# Autodesk Inventor assembly: ASSEMBLY_Main
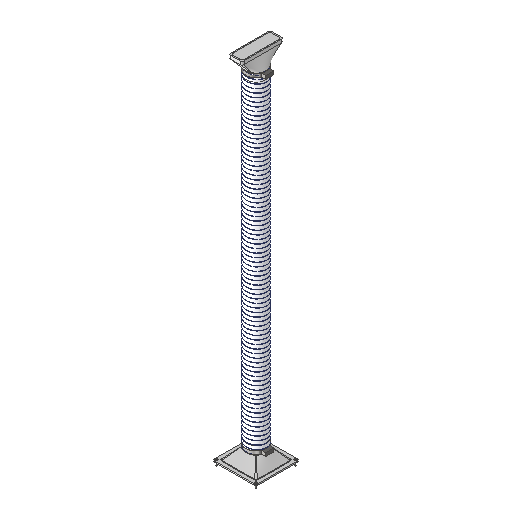
[picture p0: Inventor's stored thumbnail of the model, 512x512]
Saved by Autodesk Inventor 2025 (Build 290162010, 162A)
## iProperties
Created: 2024-10-12
Part Number: ASSEMBLY_Main
Document SubType Name: Assembly
Designer: User
Author: User
## Documents named in this file (9)
- D:\_ANDRZEJ_LACZEWSKI\_OTHER\MECH - Air Purifier Based Soldering Fume Extractor\MCAD\1_REV1\ASSEMBLY_MAIN_REVA\ASSEMBLY_Main.iam
- D:\_ANDRZEJ_LACZEWSKI\_OTHER\MECH - Air Purifier Based Soldering Fume Extractor\MCAD\1_REV1\ASSEMBLY_MAIN_REVA\3DP_PLA_Air_Purifier_60mm_Pipe_Mount.ipt
- D:\_ANDRZEJ_LACZEWSKI\_OTHER\MECH - Air Purifier Based Soldering Fume Extractor\MCAD\1_REV1\__COTS_PARTS\COTS_GENERIC_60mm_PUR_Suction_Hose.ipt
- D:\_ANDRZEJ_LACZEWSKI\_OTHER\MECH - Air Purifier Based Soldering Fume Extractor\MCAD\1_REV1\__COTS_PARTS\COTS_GENERIC_60mm_Hose_Clamp.ipt
- D:\_ANDRZEJ_LACZEWSKI\_OTHER\MECH - Air Purifier Based Soldering Fume Extractor\MCAD\1_REV1\ASSEMBLY_MAIN_REVA\3DP_PLA_Air_Funnel.ipt
- D:\_ANDRZEJ_LACZEWSKI\_OTHER\MECH - Air Purifier Based Soldering Fume Extractor\MCAD\1_REV1\ASSEMBLY_MAIN_REVA\3DP_PLA_Air_Funnel_Grid.ipt
- D:\_ANDRZEJ_LACZEWSKI\_OTHER\MECH - Air Purifier Based Soldering Fume Extractor\MCAD\1_REV1\__CONTENT_CENTER_PARTS\en-US\DIN 125-2  A\DIN 125-2 - A 3,2A.ipt
- D:\_ANDRZEJ_LACZEWSKI\_OTHER\MECH - Air Purifier Based Soldering Fume Extractor\MCAD\1_REV1\__CONTENT_CENTER_PARTS\en-US\ISO 7380-1\ISO 7380-1 - M3 x 16.ipt
- D:\_ANDRZEJ_LACZEWSKI\_OTHER\MECH - Air Purifier Based Soldering Fume Extractor\MCAD\1_REV1\__CONTENT_CENTER_PARTS\en-US\DIN 934\DIN 934 - M3 x 0,5.ipt
## Components (22 placed, 8 different names)
1. 3DP_PLA_Air_Purifier_60mm_Pipe_Mount:1 — Mate:1, Mate:4, Flush:3, Angle:1, Mate:41, Mate:42, Mate:43, Mate:44, Mate:45, Mate:46, Mate:47, Mate:48, Mate:49, Mate:50, Mate:51, Mate:52, Mate:53, Mate:54, Mate:55, Mate:56, Mate:57
2. COTS_GENERIC_60mm_PUR_Suction_Hose:1 — Mate:1, Mate:4, Mate:37, Mate:38, Flush:1, Flush:2, Mate:39, Mate:40
3. COTS_GENERIC_60mm_Hose_Clamp:1 — Mate:37, Flush:2
4. COTS_GENERIC_60mm_Hose_Clamp:2 — Mate:38, Flush:1
5. 3DP_PLA_Air_Funnel:1 — Mate:39, Mate:40, Angle:1, Flush:4
6. 3DP_PLA_Air_Funnel_Grid:1 — Flush:4
7. DIN 934 - replaced by DIN EN 24032/28673/28674 M3:4 — Insert:8
8. DIN 934 - replaced by DIN EN 24032/28673/28674 M3:3 — Insert:7
9. DIN 934 - replaced by DIN EN 24032/28673/28674 M3:2 — Insert:6
10. DIN 125-2 A A 3,2:8 — Mate:56, Mate:57, Insert:8
11. DIN 125-2 A A 3,2:7 — Mate:54, Mate:55, Insert:7
12. DIN 125-2 A A 3,2:6 — Mate:52, Mate:53, Insert:6
13. ISO 7380-1 M3 x 16:4 — Insert:4
14. ISO 7380-1 M3 x 16:3 — Insert:3
15. ISO 7380-1 M3 x 16:2 — Insert:2
16. DIN 125-2 A A 3,2:5 — Mate:48, Mate:49, Insert:4
17. DIN 125-2 A A 3,2:4 — Mate:46, Mate:47, Insert:3
18. DIN 125-2 A A 3,2:3 — Mate:44, Mate:45, Insert:2
19. DIN 934 - replaced by DIN EN 24032/28673/28674 M3:1 — Insert:5
20. DIN 125-2 A A 3,2:2 — Mate:50, Mate:51, Insert:5
21. ISO 7380-1 M3 x 16:1 — Insert:1
22. DIN 125-2 A A 3,2:1 — Mate:42, Mate:43, Insert:1
## Relationships (36: Mate 23, Insert 8, Flush 4, Angle 1)
- Mate:1: 3DP_PLA_Air_Purifier_60mm_Pipe_Mount:1 ↔ COTS_GENERIC_60mm_PUR_Suction_Hose:1
- Mate:4 (-25 mm): 3DP_PLA_Air_Purifier_60mm_Pipe_Mount:1 ↔ COTS_GENERIC_60mm_PUR_Suction_Hose:1
- Mate:37: COTS_GENERIC_60mm_PUR_Suction_Hose:1 ↔ COTS_GENERIC_60mm_Hose_Clamp:1
- Mate:38: COTS_GENERIC_60mm_PUR_Suction_Hose:1 ↔ COTS_GENERIC_60mm_Hose_Clamp:2
- Flush:1: COTS_GENERIC_60mm_PUR_Suction_Hose:1 ↔ COTS_GENERIC_60mm_Hose_Clamp:2
- Flush:2: COTS_GENERIC_60mm_PUR_Suction_Hose:1 ↔ COTS_GENERIC_60mm_Hose_Clamp:1
- Flush:3: 3DP_PLA_Air_Purifier_60mm_Pipe_Mount:1
- Mate:39: COTS_GENERIC_60mm_PUR_Suction_Hose:1 ↔ 3DP_PLA_Air_Funnel:1
- Mate:40 (-25 mm): COTS_GENERIC_60mm_PUR_Suction_Hose:1 ↔ 3DP_PLA_Air_Funnel:1
- Angle:1 (0 deg): 3DP_PLA_Air_Purifier_60mm_Pipe_Mount:1 ↔ 3DP_PLA_Air_Funnel:1
- Flush:4: 3DP_PLA_Air_Funnel:1 ↔ 3DP_PLA_Air_Funnel_Grid:1
- Mate:41 (-500 mm): 3DP_PLA_Air_Purifier_60mm_Pipe_Mount:1
- Mate:42: 3DP_PLA_Air_Purifier_60mm_Pipe_Mount:1 ↔ DIN 125-2 A A 3,2:1
- Mate:43: 3DP_PLA_Air_Purifier_60mm_Pipe_Mount:1 ↔ DIN 125-2 A A 3,2:1
- Mate:44: 3DP_PLA_Air_Purifier_60mm_Pipe_Mount:1 ↔ DIN 125-2 A A 3,2:3
- Mate:45: 3DP_PLA_Air_Purifier_60mm_Pipe_Mount:1 ↔ DIN 125-2 A A 3,2:3
- Mate:46: 3DP_PLA_Air_Purifier_60mm_Pipe_Mount:1 ↔ DIN 125-2 A A 3,2:4
- Mate:47: 3DP_PLA_Air_Purifier_60mm_Pipe_Mount:1 ↔ DIN 125-2 A A 3,2:4
- Mate:48: 3DP_PLA_Air_Purifier_60mm_Pipe_Mount:1 ↔ DIN 125-2 A A 3,2:5
- Mate:49: 3DP_PLA_Air_Purifier_60mm_Pipe_Mount:1 ↔ DIN 125-2 A A 3,2:5
- Insert:1: ISO 7380-1 M3 x 16:1 ↔ DIN 125-2 A A 3,2:1
- Insert:2: ISO 7380-1 M3 x 16:2 ↔ DIN 125-2 A A 3,2:3
- Insert:3: ISO 7380-1 M3 x 16:3 ↔ DIN 125-2 A A 3,2:4
- Insert:4: ISO 7380-1 M3 x 16:4 ↔ DIN 125-2 A A 3,2:5
- Mate:50: 3DP_PLA_Air_Purifier_60mm_Pipe_Mount:1 ↔ DIN 125-2 A A 3,2:2
- Mate:51: 3DP_PLA_Air_Purifier_60mm_Pipe_Mount:1 ↔ DIN 125-2 A A 3,2:2
- Mate:52: 3DP_PLA_Air_Purifier_60mm_Pipe_Mount:1 ↔ DIN 125-2 A A 3,2:6
- Mate:53: 3DP_PLA_Air_Purifier_60mm_Pipe_Mount:1 ↔ DIN 125-2 A A 3,2:6
- Mate:54: 3DP_PLA_Air_Purifier_60mm_Pipe_Mount:1 ↔ DIN 125-2 A A 3,2:7
- Mate:55: 3DP_PLA_Air_Purifier_60mm_Pipe_Mount:1 ↔ DIN 125-2 A A 3,2:7
- Mate:56: 3DP_PLA_Air_Purifier_60mm_Pipe_Mount:1 ↔ DIN 125-2 A A 3,2:8
- Mate:57: 3DP_PLA_Air_Purifier_60mm_Pipe_Mount:1 ↔ DIN 125-2 A A 3,2:8
- Insert:5: DIN 934 - replaced by DIN EN 24032/28673/28674 M3:1 ↔ DIN 125-2 A A 3,2:2
- Insert:6: DIN 934 - replaced by DIN EN 24032/28673/28674 M3:2 ↔ DIN 125-2 A A 3,2:6
- Insert:7: DIN 934 - replaced by DIN EN 24032/28673/28674 M3:3 ↔ DIN 125-2 A A 3,2:7
- Insert:8: DIN 934 - replaced by DIN EN 24032/28673/28674 M3:4 ↔ DIN 125-2 A A 3,2:8
